# Autodesk Inventor assembly: Montaje Bobinador
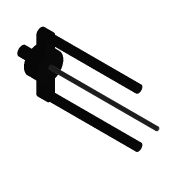
[picture p0: Inventor's stored thumbnail of the model, 180x180]
Saved by Autodesk Inventor 2022 (Build 260153000, 153)
## iProperties
Created: 2021-08-17
Part Number: Montaje Bobinador
Document SubType Name: Assembly
Designer: cristiano.schuster
Author: cristiano.schuster
## Documents named in this file (5)
- G:\Mi unidad\UTEC\Proyectos\Flor de Lana\Diseño 20191119\Montaje Bobinador.iam
- G:\Mi unidad\UTEC\Proyectos\Flor de Lana\Diseño 20191119\soporte planetario.ipt
- G:\Mi unidad\UTEC\Proyectos\Flor de Lana\Diseño 20191119\brazos_planetarios1.ipt
- G:\Mi unidad\UTEC\Proyectos\Flor de Lana\Diseño 20191119\brazos_planetarios2.ipt
- G:\Mi unidad\UTEC\Proyectos\Flor de Lana\Diseño 20191119\Varilla_Enroscada.ipt
## Components (6 placed, 4 different names)
1. soporte planetario:1 — Rigid:1, Rigid:2, Rotational:1
2. brazos_planetarios1:1 — Rigid:2, Rigid:3
3. brazos_planetarios2:1 — Rigid:3
4. brazos_planetarios1:2 — Rigid:1, Rigid:4
5. brazos_planetarios2:2 — Rigid:4
6. Varilla_Enroscada:1 — Rotational:1
## Relationships (5: WeldJoint 4, RevoluteJoint 1)
- Rigid:1 [WeldJoint]: soporte planetario:1 ↔ brazos_planetarios1:2
- Rigid:2 [WeldJoint]: soporte planetario:1 ↔ brazos_planetarios1:1
- Rigid:3 [WeldJoint]: brazos_planetarios1:1 ↔ brazos_planetarios2:1
- Rigid:4 [WeldJoint]: brazos_planetarios1:2 ↔ brazos_planetarios2:2
- Rotational:1 [RevoluteJoint] (-2 mm): soporte planetario:1 ↔ Varilla_Enroscada:1
